# Autodesk Inventor assembly: CartesianRobotWorkSpace
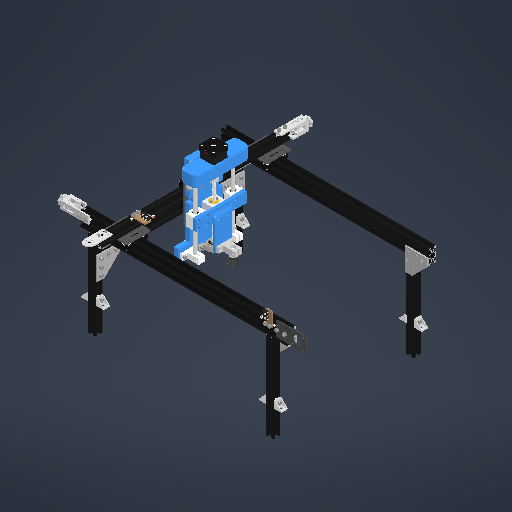
[picture p0: Inventor's stored thumbnail of the model, 512x512]
Saved by Autodesk Inventor 2027.1 (Build 311270010, 270A)
## iProperties
Created: 2026-09-29
Part Number: CartesianRobotWorkSpace
Document SubType Name: Assembly
Designer: SDS Scholar
Author: SDS Scholar
## Documents named in this file (21)
- E:\Apps\AutodeskInventor\University\MCT333_Design_of_Mechatronics_Systems_1\CAD\cartesian_robot_workspace\CartesianRobotWorkSpace.iam
- E:\Apps\AutodeskInventor\University\MCT333_Design_of_Mechatronics_Systems_1\CAD\off_the_shelf_components\AluminiumExtrusion\AluminiumExtrusion2020\Pillars.ipt
- E:\Apps\AutodeskInventor\University\MCT333_Design_of_Mechatronics_Systems_1\CAD\off_the_shelf_components\CornerBracket2020\CornerBracket2020.ipt
- C:\Users\SDS Scholar\Documents\Inventor\Content Center Files\R2027\en-US\SS-ISO 4762\ISO 4762 - M5 x 10SS-ISO.ipt
- E:\Apps\AutodeskInventor\University\MCT333_Design_of_Mechatronics_Systems_1\CAD\off_the_shelf_components\T_nuts\Slider T-Nut for 2020 - M5.ipt
- E:\Apps\AutodeskInventor\University\MCT333_Design_of_Mechatronics_Systems_1\CAD\off_the_shelf_components\RightAngleCornerPlate2020\2020 corner joining plate v1.ipt
- E:\Apps\AutodeskInventor\University\MCT333_Design_of_Mechatronics_Systems_1\CAD\off_the_shelf_components\AluminiumExtrusion\Extrusion2040\2040extrusion_ipt\X_Axis.ipt
- E:\Apps\AutodeskInventor\University\MCT333_Design_of_Mechatronics_Systems_1\CAD\off_the_shelf_components\AluminiumExtrusion\AluminiumExtrusion2020\SupportBeam.ipt
- E:\Apps\AutodeskInventor\University\MCT333_Design_of_Mechatronics_Systems_1\CAD\off_the_shelf_components\VSoltGantrySetAllSizes\20mm Gantry Set\20mm Gantry Set.ipt
- E:\Apps\AutodeskInventor\University\MCT333_Design_of_Mechatronics_Systems_1\CAD\off_the_shelf_components\RightAngleCornerPlate2020\2020 corner joining plate v1_MIR2.ipt
- E:\Apps\AutodeskInventor\University\MCT333_Design_of_Mechatronics_Systems_1\CAD\off_the_shelf_components\T_nuts\Slider T-Nut for 2020 - M5_MIR2.ipt
- E:\Apps\AutodeskInventor\University\MCT333_Design_of_Mechatronics_Systems_1\CAD\off_the_shelf_components\nema-17-23-stepper-motor-mounts\NEMA 17 Flat.ipt
- E:\Apps\AutodeskInventor\University\MCT333_Design_of_Mechatronics_Systems_1\CAD\off_the_shelf_components\GT2BeltTensioner\2020 Belt Tensioner G_K.ipt
- E:\Apps\AutodeskInventor\University\MCT333_Design_of_Mechatronics_Systems_1\CAD\cartesian_robot_workspace\Y_Axis.iam
- E:\Apps\AutodeskInventor\University\MCT333_Design_of_Mechatronics_Systems_1\CAD\cartesian_robot_workspace\Z Axis\Z-Axis.iam
- E:\Apps\AutodeskInventor\University\MCT333_Design_of_Mechatronics_Systems_1\CAD\cartesian_robot_workspace\LimitSwitchMountPlate.ipt
- E:\Apps\AutodeskInventor\University\MCT333_Design_of_Mechatronics_Systems_1\CAD\off_the_shelf_components\T_nuts\Slider T-Nut for 2020 - M3.ipt
- E:\Apps\AutodeskInventor\University\MCT333_Design_of_Mechatronics_Systems_1\CAD\electronic_components\NO-NC Bump Switch\NO-NC Bump Switch.ipt
- C:\Users\SDS Scholar\Documents\Inventor\Content Center Files\R2027\en-US\DIN 7985 (H)\DIN 7985 (H) - M2.5x12-H.ipt
- C:\Users\SDS Scholar\Documents\Inventor\Content Center Files\R2027\en-US\ISO 4032(2)\ISO 4032 - M2.5 - ISO.ipt
- E:\Apps\AutodeskInventor\University\MCT333_Design_of_Mechatronics_Systems_1\CAD\DESIGN1_CAD_parameters.xlsx
## Components (125 placed, 19 different names)
1. Z-Axis:1 [sub-assembly] — Tangent:9, Tangent:10, Mate:231, Mate:232
2. Slider T-Nut for 2020 - M3:1 — Mate:234, Mate:235, Mate:239
3. Slider T-Nut for 2020 - M3:2 — Mate:236, Mate:237, Mate:242
4. SS ISO 4762 M5 x 10:70 — Mate:239, Mate:240, Mate:255
5. SS ISO 4762 M5 x 10:71 — Mate:242, Mate:243, Mate:254
6. DIN 7985 (H) M2.5x12-H:1 — Mate:251, Mate:258, Mate:260, Mate:263
7. DIN 7985 (H) M2.5x12-H:2 — Mate:253, Mate:257, Mate:259, Mate:262
8. ISO 4032 M2.5:1 — Mate:251, Mate:265
9. ISO 4032 M2.5:2 — Mate:253, Mate:264
10. NO-NC Bump Switch:1 — Mate:257, Mate:258, Mate:261, Mate:262, Mate:263
11. LimitSwitchMountPlate:1 — Mate:254, Mate:255, Mate:256, Mate:259, Mate:260, Mate:261, Mate:264, Mate:265, Flush:194
12. SupportBeam:1 — Mate:123, Mate:124, Mate:125, Mate:126, Mate:138, Mate:141, Mate:143, Mate:202
13. X_Axis:1 — Mate:32, Mate:33, Mate:34, Mate:35, Mate:36, Mate:37, Mate:48, Mate:49, Mate:56, Mate:59, Flush:3, Tangent:1, Tangent:2, Mate:145, Mate:146, Mate:147, Mate:148, Mate:151, Mate:154, Mate:155, Flush:6, Mate:156, Mate:157, Mate:158, Mate:159, Mate:162, Mate:165, Mate:217, Mate:228, Flush:193, Mate:234, Mate:235, Mate:236, Mate:237, Mate:240, Mate:243, Mate:256
14. X_Axis:2 — Mate:89, Mate:90, Mate:91, Mate:92, Mate:93, Mate:94, Mate:107, Mate:110, Mate:113, Mate:115, Flush:4, Tangent:5, Tangent:6, Mate:225
15. NEMA 17 Flat:1 — Mate:149, Mate:152, Mate:155
16. Slider T-Nut for 2020 - M5:40 — Mate:145, Mate:146, Mate:150, Flush:6
17. Slider T-Nut for 2020 - M5:41 — Mate:147, Mate:148, Mate:153
18. SS ISO 4762 M5 x 10:58 — Mate:149, Mate:150, Mate:151
19. SS ISO 4762 M5 x 10:59 — Mate:152, Mate:153, Mate:154
20. 2020 Belt Tensioner G_K:1 — Mate:226, Mate:227, Mate:228
21. Slider T-Nut for 2020 - M5:42 — Mate:156, Mate:157, Mate:161, Mate:179, Flush:193
22. Slider T-Nut for 2020 - M5:43 — Mate:158, Mate:159, Mate:164
23. SS ISO 4762 M5 x 10:60 — Mate:164, Mate:165, Mate:227
24. SS ISO 4762 M5 x 10:61 — Mate:161, Mate:162, Mate:179, Mate:226
25. 20mm Gantry Set:1 — Tangent:1, Tangent:2, Flush:5, Mate:171, Flush:9, Mate:229, Mate:230
26. 20mm Gantry Set:2 — Tangent:5, Tangent:6, Flush:5, Mate:174, Mate:177, Flush:8, Flush:9, Mate:232
27. Y_Axis:1 [sub-assembly] — Mate:167, Mate:168, Mate:169, Mate:170, Mate:173, Mate:176, Mate:177, Flush:8, Tangent:9, Tangent:10, Mate:231
28. Slider T-Nut for 2020 - M5:44 — Mate:167, Mate:168, Mate:172
29. Slider T-Nut for 2020 - M5:45 — Mate:169, Mate:170, Mate:175
30. SS ISO 4762 M5 x 10:62 — Mate:174, Mate:175, Mate:176
31. SS ISO 4762 M5 x 10:63 — Mate:171, Mate:172, Mate:173
32. Pillars:1 — Flush:10, Flush:11, Mate:183, Mate:184, Mate:185, Mate:186, Mate:187, Mate:188, Mate:189, Flush:191, Flush:192, Mate:190, Symmetry:1, Mate:191, Mate:192, Mate:193, Mate:194, Mate:195, Mate:196, Mate:197, Mate:198, Mate:199, Mate:200, Mate:201, Mate:202
33. SS ISO 4762 M5 x 10:2 — Mate:28, Mate:29, Mate:189
34. Slider T-Nut for 2020 - M5:2 — Mate:29, Mate:186, Mate:187
35. Slider T-Nut for 2020 - M5:1 — Mate:21, Mate:184, Mate:185
36. SS ISO 4762 M5 x 10:1 — Mate:20, Mate:21, Mate:31, Mate:188
37. CornerBracket2020:1 — Mate:20, Mate:31, Flush:191
38. CornerBracket2020:4 — Mate:28, Flush:192, Mate:190
39. Pillars:2 — Mate:218, Mate:219, Mate:220, Mate:221, Mate:222, Mate:223, Mate:224, Mate:225
40. SS ISO 4762 M5 x 10:64
41. Slider T-Nut for 2020 - M5:46
42. Slider T-Nut for 2020 - M5:47
43. SS ISO 4762 M5 x 10:65
44. CornerBracket2020:5
45. CornerBracket2020:6
46. Pillars:3 — Symmetry:1
47. SS ISO 4762 M5 x 10:66
48. Slider T-Nut for 2020 - M5:48
49. Slider T-Nut for 2020 - M5:49
50. SS ISO 4762 M5 x 10:67
51. CornerBracket2020:7
52. CornerBracket2020:8
53. Pillars:4 — Mate:210, Mate:211, Mate:212, Mate:213, Mate:214, Mate:215, Mate:216, Mate:217
54. SS ISO 4762 M5 x 10:68
55. Slider T-Nut for 2020 - M5:50
56. Slider T-Nut for 2020 - M5:51
57. SS ISO 4762 M5 x 10:69
58. CornerBracket2020:9
59. CornerBracket2020:10
60. 2020 corner joining plate v1:6 — Mate:127, Mate:130, Mate:133, Mate:136, Mate:139, Mate:143, Mate:144, Mate:201
61. Slider T-Nut for 2020 - M5:35 — Mate:131, Mate:192, Mate:195
62. Slider T-Nut for 2020 - M5:36 — Mate:123, Mate:124, Mate:137
63. Slider T-Nut for 2020 - M5:37 — Mate:134, Mate:191, Mate:194, Mate:196
64. Slider T-Nut for 2020 - M5:38 — Mate:125, Mate:126, Mate:140
65. Slider T-Nut for 2020 - M5:39 — Mate:128, Mate:193, Mate:197
66. SS ISO 4762 M5 x 10:48 — Mate:127, Mate:128, Mate:198
67. SS ISO 4762 M5 x 10:49 — Mate:139, Mate:140, Mate:141
68. SS ISO 4762 M5 x 10:50 — Mate:130, Mate:131, Mate:199
69. SS ISO 4762 M5 x 10:51 — Mate:133, Mate:134, Mate:200
70. SS ISO 4762 M5 x 10:52 — Mate:136, Mate:137, Mate:138
71. 2020 corner joining plate v1_MIR2:1
72. Slider T-Nut for 2020 - M5_MIR2:1
73. Slider T-Nut for 2020 - M5_MIR2:2
74. Slider T-Nut for 2020 - M5_MIR2:3
75. Slider T-Nut for 2020 - M5_MIR2:4
76. Slider T-Nut for 2020 - M5_MIR2:5
77. SS ISO 4762 M5 x 10:53
78. SS ISO 4762 M5 x 10:54
79. SS ISO 4762 M5 x 10:55
80. SS ISO 4762 M5 x 10:56
81. SS ISO 4762 M5 x 10:57
82. 2020 corner joining plate v1:1 — Mate:42, Mate:46, Mate:49, Mate:51, Mate:54, Mate:57, Flush:3, Mate:216, Mate:230, Flush:194
83. Slider T-Nut for 2020 - M5:9 — Mate:36, Mate:37, Mate:55
84. Slider T-Nut for 2020 - M5:10 — Mate:52, Mate:212, Mate:213
85. Slider T-Nut for 2020 - M5:11 — Mate:43, Mate:210, Mate:211
86. Slider T-Nut for 2020 - M5:12 — Mate:34, Mate:35, Mate:58
87. Slider T-Nut for 2020 - M5:13 — Mate:32, Mate:33, Mate:47
88. SS ISO 4762 M5 x 10:9 — Mate:42, Mate:43, Mate:215
89. SS ISO 4762 M5 x 10:10 — Mate:46, Mate:47, Mate:48
90. SS ISO 4762 M5 x 10:11 — Mate:54, Mate:55, Mate:56
91. SS ISO 4762 M5 x 10:12 — Mate:51, Mate:52, Mate:214
92. SS ISO 4762 M5 x 10:13 — Mate:57, Mate:58, Mate:59
93. 2020 corner joining plate v1:2 — Mate:229
94. Slider T-Nut for 2020 - M5:14
95. Slider T-Nut for 2020 - M5:15
96. Slider T-Nut for 2020 - M5:16
97. Slider T-Nut for 2020 - M5:17
98. Slider T-Nut for 2020 - M5:18
99. SS ISO 4762 M5 x 10:14
100. SS ISO 4762 M5 x 10:15
101. SS ISO 4762 M5 x 10:16
102. SS ISO 4762 M5 x 10:17
103. SS ISO 4762 M5 x 10:18
104. 2020 corner joining plate v1:4 — Mate:99, Mate:102, Mate:105, Mate:108, Mate:111, Mate:115, Flush:4, Mate:224
105. Slider T-Nut for 2020 - M5:25 — Mate:93, Mate:94, Mate:106
106. Slider T-Nut for 2020 - M5:26 — Mate:103, Mate:218, Mate:219
107. Slider T-Nut for 2020 - M5:27 — Mate:100, Mate:220, Mate:221
108. Slider T-Nut for 2020 - M5:28 — Mate:91, Mate:92, Mate:109
109. Slider T-Nut for 2020 - M5:29 — Mate:89, Mate:90, Mate:112
110. SS ISO 4762 M5 x 10:38 — Mate:99, Mate:100, Mate:223
111. SS ISO 4762 M5 x 10:39 — Mate:105, Mate:106, Mate:107
112. SS ISO 4762 M5 x 10:40 — Mate:102, Mate:103, Mate:222
113. SS ISO 4762 M5 x 10:41 — Mate:108, Mate:109, Mate:110
114. SS ISO 4762 M5 x 10:42 — Mate:111, Mate:112, Mate:113
115. 2020 corner joining plate v1:5 — Mate:144
116. Slider T-Nut for 2020 - M5:30
117. Slider T-Nut for 2020 - M5:31
118. Slider T-Nut for 2020 - M5:32
119. Slider T-Nut for 2020 - M5:33
120. Slider T-Nut for 2020 - M5:34
121. SS ISO 4762 M5 x 10:43
122. SS ISO 4762 M5 x 10:44
123. SS ISO 4762 M5 x 10:45
124. SS ISO 4762 M5 x 10:46
125. SS ISO 4762 M5 x 10:47
## Component patterns: (4 elements, first: Pillars:1 + SS ISO 4762 M5 x 10:2 + Slider T-Nut for 2020 - M5:2 + Slider T-Nut for 2020 - M5:1 + SS ISO 4762 M5 x 10:1 + CornerBracket2020:1 + CornerBracket2020:4), (2 elements, first: 2020 corner joining plate v1:6 + Slider T-Nut for 2020 - M5:35 + Slider T-Nut for 2020 - M5:36 + Slider T-Nut for 2020 - M5:37 + Slider T-Nut for 2020 - M5:38 + Slider T-Nut for 2020 - M5:39 + SS ISO 4762 M5 x 10:48 + SS ISO 4762 M5 x 10:49 + SS ISO 4762 M5 x 10:50 + SS ISO 4762 M5 x 10:51 + SS ISO 4762 M5 x 10:52), (2 elements, first: 2020 corner joining plate v1:1 + Slider T-Nut for 2020 - M5:9 + Slider T-Nut for 2020 - M5:10 + Slider T-Nut for 2020 - M5:11 + Slider T-Nut for 2020 - M5:12 + Slider T-Nut for 2020 - M5:13 + SS ISO 4762 M5 x 10:9 + SS ISO 4762 M5 x 10:10 + SS ISO 4762 M5 x 10:11 + SS ISO 4762 M5 x 10:12 + SS ISO 4762 M5 x 10:13), (2 elements, first: 2020 corner joining plate v1:4 + Slider T-Nut for 2020 - M5:25 + Slider T-Nut for 2020 - M5:26 + Slider T-Nut for 2020 - M5:27 + Slider T-Nut for 2020 - M5:28 + Slider T-Nut for 2020 - M5:29 + SS ISO 4762 M5 x 10:38 + SS ISO 4762 M5 x 10:39 + SS ISO 4762 M5 x 10:40 + SS ISO 4762 M5 x 10:41 + SS ISO 4762 M5 x 10:42)
## Relationships (178: Mate 159, Flush 12, Tangent 6, Symmetry 1)
- Mate:20: SS ISO 4762 M5 x 10:1 ↔ CornerBracket2020:1
- Mate:21: Slider T-Nut for 2020 - M5:1 ↔ SS ISO 4762 M5 x 10:1
- Mate:28: SS ISO 4762 M5 x 10:2 ↔ CornerBracket2020:4
- Mate:29: SS ISO 4762 M5 x 10:2 ↔ Slider T-Nut for 2020 - M5:2
- Mate:31 (0.7 mm): SS ISO 4762 M5 x 10:1 ↔ CornerBracket2020:1
- Mate:32: X_Axis:1 ↔ Slider T-Nut for 2020 - M5:13
- Mate:33: X_Axis:1 ↔ Slider T-Nut for 2020 - M5:13
- Mate:34: X_Axis:1 ↔ Slider T-Nut for 2020 - M5:12
- Mate:35: X_Axis:1 ↔ Slider T-Nut for 2020 - M5:12
- Mate:36: X_Axis:1 ↔ Slider T-Nut for 2020 - M5:9
- Mate:37: X_Axis:1 ↔ Slider T-Nut for 2020 - M5:9
- Mate:42: 2020 corner joining plate v1:1 ↔ SS ISO 4762 M5 x 10:9
- Mate:43: Slider T-Nut for 2020 - M5:11 ↔ SS ISO 4762 M5 x 10:9
- Mate:46: 2020 corner joining plate v1:1 ↔ SS ISO 4762 M5 x 10:10
- Mate:47: Slider T-Nut for 2020 - M5:13 ↔ SS ISO 4762 M5 x 10:10
- Mate:48: X_Axis:1 ↔ SS ISO 4762 M5 x 10:10
- Mate:49: X_Axis:1 ↔ 2020 corner joining plate v1:1
- Mate:51: 2020 corner joining plate v1:1 ↔ SS ISO 4762 M5 x 10:12
- Mate:52: Slider T-Nut for 2020 - M5:10 ↔ SS ISO 4762 M5 x 10:12
- Mate:54: 2020 corner joining plate v1:1 ↔ SS ISO 4762 M5 x 10:11
- Mate:55: Slider T-Nut for 2020 - M5:9 ↔ SS ISO 4762 M5 x 10:11
- Mate:56: X_Axis:1 ↔ SS ISO 4762 M5 x 10:11
- Mate:57: 2020 corner joining plate v1:1 ↔ SS ISO 4762 M5 x 10:13
- Mate:58: Slider T-Nut for 2020 - M5:12 ↔ SS ISO 4762 M5 x 10:13
- Mate:59: X_Axis:1 ↔ SS ISO 4762 M5 x 10:13
- Flush:3: X_Axis:1 ↔ 2020 corner joining plate v1:1
- Tangent:1: X_Axis:1 ↔ 20mm Gantry Set:1
- Tangent:2: X_Axis:1 ↔ 20mm Gantry Set:1
- Mate:89: X_Axis:2 ↔ Slider T-Nut for 2020 - M5:29
- Mate:90: X_Axis:2 ↔ Slider T-Nut for 2020 - M5:29
- Mate:91: X_Axis:2 ↔ Slider T-Nut for 2020 - M5:28
- Mate:92: X_Axis:2 ↔ Slider T-Nut for 2020 - M5:28
- Mate:93: X_Axis:2 ↔ Slider T-Nut for 2020 - M5:25
- Mate:94: X_Axis:2 ↔ Slider T-Nut for 2020 - M5:25
- Mate:99: 2020 corner joining plate v1:4 ↔ SS ISO 4762 M5 x 10:38
- Mate:100: Slider T-Nut for 2020 - M5:27 ↔ SS ISO 4762 M5 x 10:38
- Mate:102: 2020 corner joining plate v1:4 ↔ SS ISO 4762 M5 x 10:40
- Mate:103: Slider T-Nut for 2020 - M5:26 ↔ SS ISO 4762 M5 x 10:40
- Mate:105: 2020 corner joining plate v1:4 ↔ SS ISO 4762 M5 x 10:39
- Mate:106: Slider T-Nut for 2020 - M5:25 ↔ SS ISO 4762 M5 x 10:39
- Mate:107: X_Axis:2 ↔ SS ISO 4762 M5 x 10:39
- Mate:108: 2020 corner joining plate v1:4 ↔ SS ISO 4762 M5 x 10:41
- Mate:109: Slider T-Nut for 2020 - M5:28 ↔ SS ISO 4762 M5 x 10:41
- Mate:110: X_Axis:2 ↔ SS ISO 4762 M5 x 10:41
- Mate:111: 2020 corner joining plate v1:4 ↔ SS ISO 4762 M5 x 10:42
- Mate:112: Slider T-Nut for 2020 - M5:29 ↔ SS ISO 4762 M5 x 10:42
- Mate:113: X_Axis:2 ↔ SS ISO 4762 M5 x 10:42
- Mate:115: X_Axis:2 ↔ 2020 corner joining plate v1:4
- Flush:4: X_Axis:2 ↔ 2020 corner joining plate v1:4
- Mate:123: SupportBeam:1 ↔ Slider T-Nut for 2020 - M5:36
- Mate:124: SupportBeam:1 ↔ Slider T-Nut for 2020 - M5:36
- Mate:125: SupportBeam:1 ↔ Slider T-Nut for 2020 - M5:38
- Mate:126: SupportBeam:1 ↔ Slider T-Nut for 2020 - M5:38
- Mate:127: 2020 corner joining plate v1:6 ↔ SS ISO 4762 M5 x 10:48
- Mate:128: Slider T-Nut for 2020 - M5:39 ↔ SS ISO 4762 M5 x 10:48
- Mate:130: 2020 corner joining plate v1:6 ↔ SS ISO 4762 M5 x 10:50
- Mate:131: Slider T-Nut for 2020 - M5:35 ↔ SS ISO 4762 M5 x 10:50
- Mate:133: 2020 corner joining plate v1:6 ↔ SS ISO 4762 M5 x 10:51
- Mate:134: Slider T-Nut for 2020 - M5:37 ↔ SS ISO 4762 M5 x 10:51
- Mate:136: 2020 corner joining plate v1:6 ↔ SS ISO 4762 M5 x 10:52
- Mate:137: Slider T-Nut for 2020 - M5:36 ↔ SS ISO 4762 M5 x 10:52
- Mate:138: SupportBeam:1 ↔ SS ISO 4762 M5 x 10:52
- Mate:139: 2020 corner joining plate v1:6 ↔ SS ISO 4762 M5 x 10:49
- Mate:140: Slider T-Nut for 2020 - M5:38 ↔ SS ISO 4762 M5 x 10:49
- Mate:141: SupportBeam:1 ↔ SS ISO 4762 M5 x 10:49
- Mate:143: SupportBeam:1 ↔ 2020 corner joining plate v1:6
- Mate:144 (5 mm): 2020 corner joining plate v1:6 ↔ 2020 corner joining plate v1:5
- Tangent:5: X_Axis:2 ↔ 20mm Gantry Set:2
- Tangent:6: X_Axis:2 ↔ 20mm Gantry Set:2
- Flush:5: 20mm Gantry Set:1 ↔ 20mm Gantry Set:2
- Mate:145: X_Axis:1 ↔ Slider T-Nut for 2020 - M5:40
- Mate:146: X_Axis:1 ↔ Slider T-Nut for 2020 - M5:40
- Mate:147: X_Axis:1 ↔ Slider T-Nut for 2020 - M5:41
- Mate:148: X_Axis:1 ↔ Slider T-Nut for 2020 - M5:41
- Mate:149: NEMA 17 Flat:1 ↔ SS ISO 4762 M5 x 10:58
- Mate:150: Slider T-Nut for 2020 - M5:40 ↔ SS ISO 4762 M5 x 10:58
- Mate:151: X_Axis:1 ↔ SS ISO 4762 M5 x 10:58
- Mate:152: NEMA 17 Flat:1 ↔ SS ISO 4762 M5 x 10:59
- Mate:153: Slider T-Nut for 2020 - M5:41 ↔ SS ISO 4762 M5 x 10:59
- Mate:154: X_Axis:1 ↔ SS ISO 4762 M5 x 10:59
- Mate:155: X_Axis:1 ↔ NEMA 17 Flat:1
- Flush:6: X_Axis:1 ↔ Slider T-Nut for 2020 - M5:40
- Mate:156: X_Axis:1 ↔ Slider T-Nut for 2020 - M5:42
- Mate:157: X_Axis:1 ↔ Slider T-Nut for 2020 - M5:42
- Mate:158: X_Axis:1 ↔ Slider T-Nut for 2020 - M5:43
- Mate:159: X_Axis:1 ↔ Slider T-Nut for 2020 - M5:43
- Mate:161: Slider T-Nut for 2020 - M5:42 ↔ SS ISO 4762 M5 x 10:61
- Mate:162: X_Axis:1 ↔ SS ISO 4762 M5 x 10:61
- Mate:164: Slider T-Nut for 2020 - M5:43 ↔ SS ISO 4762 M5 x 10:60
- Mate:165: X_Axis:1 ↔ SS ISO 4762 M5 x 10:60
- Mate:167: Y_Axis:1 ↔ Slider T-Nut for 2020 - M5:44
- Mate:168: Y_Axis:1 ↔ Slider T-Nut for 2020 - M5:44
- Mate:169: Y_Axis:1 ↔ Slider T-Nut for 2020 - M5:45
- Mate:170: Y_Axis:1 ↔ Slider T-Nut for 2020 - M5:45
- Mate:171: 20mm Gantry Set:1 ↔ SS ISO 4762 M5 x 10:63
- Mate:172: Slider T-Nut for 2020 - M5:44 ↔ SS ISO 4762 M5 x 10:63
- Mate:173: Y_Axis:1 ↔ SS ISO 4762 M5 x 10:63
- Mate:174: 20mm Gantry Set:2 ↔ SS ISO 4762 M5 x 10:62
- Mate:175: Slider T-Nut for 2020 - M5:45 ↔ SS ISO 4762 M5 x 10:62
- Mate:176: Y_Axis:1 ↔ SS ISO 4762 M5 x 10:62
- Mate:177: 20mm Gantry Set:2 ↔ Y_Axis:1
- Flush:8 (-20 mm): 20mm Gantry Set:2 ↔ Y_Axis:1
- Flush:9: 20mm Gantry Set:1 ↔ 20mm Gantry Set:2
- Mate:179: Slider T-Nut for 2020 - M5:42 ↔ SS ISO 4762 M5 x 10:61
- Flush:10: Pillars:1
- Flush:11: Pillars:1
- Mate:183: Pillars:1
- Mate:184: Pillars:1 ↔ Slider T-Nut for 2020 - M5:1
- Mate:185: Pillars:1 ↔ Slider T-Nut for 2020 - M5:1
- Mate:186: Pillars:1 ↔ Slider T-Nut for 2020 - M5:2
- Mate:187: Pillars:1 ↔ Slider T-Nut for 2020 - M5:2
- Mate:188: Pillars:1 ↔ SS ISO 4762 M5 x 10:1
- Mate:189: Pillars:1 ↔ SS ISO 4762 M5 x 10:2
- Flush:191 (70 mm): Pillars:1 ↔ CornerBracket2020:1
- Flush:192 (70 mm): Pillars:1 ↔ CornerBracket2020:4
- Mate:190: Pillars:1 ↔ CornerBracket2020:4
- Symmetry:1: Pillars:1 ↔ Pillars:3
- Mate:191: Pillars:1 ↔ Slider T-Nut for 2020 - M5:37
- Mate:192: Pillars:1 ↔ Slider T-Nut for 2020 - M5:35
- Mate:193: Pillars:1 ↔ Slider T-Nut for 2020 - M5:39
- Mate:194: Pillars:1 ↔ Slider T-Nut for 2020 - M5:37
- Mate:195: Pillars:1 ↔ Slider T-Nut for 2020 - M5:35
- Mate:196: Pillars:1 ↔ Slider T-Nut for 2020 - M5:37
- Mate:197: Pillars:1 ↔ Slider T-Nut for 2020 - M5:39
- Mate:198: Pillars:1 ↔ SS ISO 4762 M5 x 10:48
- Mate:199: Pillars:1 ↔ SS ISO 4762 M5 x 10:50
- Mate:200: Pillars:1 ↔ SS ISO 4762 M5 x 10:51
- Mate:201: Pillars:1 ↔ 2020 corner joining plate v1:6
- Mate:202: SupportBeam:1 ↔ Pillars:1
- Mate:210: Pillars:4 ↔ Slider T-Nut for 2020 - M5:11
- Mate:211: Pillars:4 ↔ Slider T-Nut for 2020 - M5:11
- Mate:212: Pillars:4 ↔ Slider T-Nut for 2020 - M5:10
- Mate:213: Pillars:4 ↔ Slider T-Nut for 2020 - M5:10
- Mate:214: Pillars:4 ↔ SS ISO 4762 M5 x 10:12
- Mate:215: Pillars:4 ↔ SS ISO 4762 M5 x 10:9
- Mate:216: Pillars:4 ↔ 2020 corner joining plate v1:1
- Mate:217: X_Axis:1 ↔ Pillars:4
- Mate:218: Pillars:2 ↔ Slider T-Nut for 2020 - M5:26
- Mate:219: Pillars:2 ↔ Slider T-Nut for 2020 - M5:26
- Mate:220: Pillars:2 ↔ Slider T-Nut for 2020 - M5:27
- Mate:221: Pillars:2 ↔ Slider T-Nut for 2020 - M5:27
- Mate:222: Pillars:2 ↔ SS ISO 4762 M5 x 10:40
- Mate:223: Pillars:2 ↔ SS ISO 4762 M5 x 10:38
- Mate:224: Pillars:2 ↔ 2020 corner joining plate v1:4
- Mate:225: X_Axis:2 ↔ Pillars:2
- Mate:226: 2020 Belt Tensioner G_K:1 ↔ SS ISO 4762 M5 x 10:61
- Mate:227: 2020 Belt Tensioner G_K:1 ↔ SS ISO 4762 M5 x 10:60
- Mate:228: X_Axis:1 ↔ 2020 Belt Tensioner G_K:1
- Flush:193: X_Axis:1 ↔ Slider T-Nut for 2020 - M5:42
- Tangent:9: Z-Axis:1 ↔ Y_Axis:1
- Tangent:10: Z-Axis:1 ↔ Y_Axis:1
- Mate:229: 20mm Gantry Set:1 ↔ 2020 corner joining plate v1:2
- Mate:230: 20mm Gantry Set:1 ↔ 2020 corner joining plate v1:1
- Mate:231: Z-Axis:1 ↔ Y_Axis:1
- Mate:232: Z-Axis:1 ↔ 20mm Gantry Set:2
- Mate:234: Slider T-Nut for 2020 - M3:1 ↔ X_Axis:1
- Mate:235: Slider T-Nut for 2020 - M3:1 ↔ X_Axis:1
- Mate:236: Slider T-Nut for 2020 - M3:2 ↔ X_Axis:1
- Mate:237: Slider T-Nut for 2020 - M3:2 ↔ X_Axis:1
- Mate:239: Slider T-Nut for 2020 - M3:1 ↔ SS ISO 4762 M5 x 10:70
- Mate:240: SS ISO 4762 M5 x 10:70 ↔ X_Axis:1
- Mate:242: Slider T-Nut for 2020 - M3:2 ↔ SS ISO 4762 M5 x 10:71
- Mate:243: SS ISO 4762 M5 x 10:71 ↔ X_Axis:1
- Mate:251: DIN 7985 (H) M2.5x12-H:1 ↔ ISO 4032 M2.5:1
- Mate:253: DIN 7985 (H) M2.5x12-H:2 ↔ ISO 4032 M2.5:2
- Mate:254: SS ISO 4762 M5 x 10:71 ↔ LimitSwitchMountPlate:1
- Mate:255: SS ISO 4762 M5 x 10:70 ↔ LimitSwitchMountPlate:1
- Mate:256: LimitSwitchMountPlate:1 ↔ X_Axis:1
- Mate:257: DIN 7985 (H) M2.5x12-H:2 ↔ NO-NC Bump Switch:1
- Mate:258: DIN 7985 (H) M2.5x12-H:1 ↔ NO-NC Bump Switch:1
- Mate:259: DIN 7985 (H) M2.5x12-H:2 ↔ LimitSwitchMountPlate:1
- Mate:260: DIN 7985 (H) M2.5x12-H:1 ↔ LimitSwitchMountPlate:1
- Mate:261: NO-NC Bump Switch:1 ↔ LimitSwitchMountPlate:1
- Mate:262: DIN 7985 (H) M2.5x12-H:2 ↔ NO-NC Bump Switch:1
- Mate:263: DIN 7985 (H) M2.5x12-H:1 ↔ NO-NC Bump Switch:1
- Mate:264: ISO 4032 M2.5:2 ↔ LimitSwitchMountPlate:1
- Mate:265: ISO 4032 M2.5:1 ↔ LimitSwitchMountPlate:1
- Flush:194: LimitSwitchMountPlate:1 ↔ 2020 corner joining plate v1:1
## Named parameters: Product_dia = 50 mm, ProductBaseHeight = 40 mm, ProductLedHeight = 20 mm, GridProcutClearance = 3 mm, GridBorderThickness = 5 mm, GridBorderFillets = 7 mm, GridTotalSize = 63 mm, GridRobotClearance = 50 mm, AluminiumExtrusionBase = 20 mm, AluminiumExtrusionClearance = 30 mm, BaseTotalWidth = 652 mm, FeedingAreaLength = 300 mm, BaseTotalLength = 812 mm, DistanceBetweenGrid = 5 mm, WorkspaceLength = 552 mm, WorkspaceWidth = 372 mm, WorkspaceHeight = 166.5 mm, AxesBaseFillet = 15 mm, Zaxis = 223 mm, ProductTotalHeight = 45 mm, VerticalClearance = 10 mm, VerticalStroke = 85 mm, FrontArea = 50 mm, BackArea = 150 mm, CylinderStroke = 75 mm, SideAreaWidth = 200 mm, BaseHeight = 70 mm, ContolBoxLength = 160 mm, DistanceBetweenBoxes = 30 mm, BoxesWidth = 140 mm, PowerBoxLength = 300 mm, PneumaticBoxLength = 200 mm, BoxesClearance = 30 mm, BoxesHeight = 170 mm, ContolBoxWidth = 250 mm, ControlBoxHeight = 120 mm, BaseWoodThickness = 7 mm, kerf = 1.5 mm, Kerf = 2 mm, TransmitterAreaWidth = 100 mm, RxThickness = 1 mm
